# Autodesk Inventor assembly: robot_over_all5
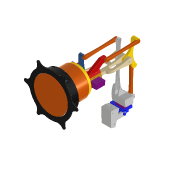
[picture p0: Inventor's stored thumbnail of the model, 180x180]
Saved by Autodesk Inventor 2022.6 (Build 266554000, 554)
## iProperties
Created: 2025-03-10
Part Number: robot_over_all5
Document SubType Name: Assembly
Designer: rugby
Author: rugby
## Documents named in this file (21)
- C:\Users\rugby\Desktop\パンケーキFA工場\ロボットアーム_機械設計\垂直多関節リンクロボット\robot_over_all5.iam
- C:\Users\rugby\Desktop\パンケーキFA工場\ロボットアーム_機械設計\垂直多関節リンクロボット\base\base_02.ipt
- C:\Users\rugby\Desktop\パンケーキFA工場\ロボットアーム_機械設計\垂直多関節リンクロボット\base\base_holderTamTam_02.ipt
- C:\Users\rugby\Desktop\パンケーキFA工場\ロボットアーム_機械設計\ServoMotor(20kg・cm)\ServoMotor(20kg・cm).ipt
- C:\Users\rugby\Desktop\パンケーキFA工場\ロボットアーム_機械設計\垂直多関節リンクロボット\base\roofparts_support_upper2.ipt
- C:\Users\rugby\Desktop\パンケーキFA工場\ロボットアーム_機械設計\垂直多関節リンクロボット\base\joint1_roofparts.ipt
- C:\Users\rugby\Desktop\パンケーキFA工場\ロボットアーム_機械設計\ServoMotor(20kg・cm)\ServoMotor_Hone1.ipt
- C:\Users\rugby\Desktop\パンケーキFA工場\ロボットアーム_機械設計\垂直多関節リンクロボット\base\j2_j3_support3.ipt
- C:\Users\rugby\Desktop\パンケーキFA工場\平行リンクロボットCAD\servo_cover2.ipt
- C:\Users\rugby\Desktop\パンケーキFA工場\ロボットアーム_機械設計\垂直多関節リンクロボット\link\arm_42.ipt
- C:\Users\rugby\Desktop\パンケーキFA工場\ロボットアーム_機械設計\ServoMotor(20kg・cm)\ServoMotor_Hone2.ipt
- C:\Users\rugby\Desktop\パンケーキFA工場\ロボットアーム_機械設計\垂直多関節リンクロボット\link\arm_53.ipt
- C:\Users\rugby\Desktop\パンケーキFA工場\ロボットアーム_機械設計\垂直多関節リンクロボット\link\arm_51.ipt
- C:\Users\rugby\Desktop\パンケーキFA工場\ロボットアーム_機械設計\垂直多関節リンクロボット\link\arm_64.ipt
- C:\Users\rugby\Desktop\パンケーキFA工場\ロボットアーム_機械設計\垂直多関節リンクロボット\link\arm_55.ipt
- C:\Users\rugby\Desktop\パンケーキFA工場\ロボットアーム_機械設計\垂直多関節リンクロボット\link\arm_63.ipt
- C:\Users\rugby\Desktop\パンケーキFA工場\ロボットアーム_機械設計\垂直多関節リンクロボット\wrist1\j4_cover 2.ipt
- C:\Users\rugby\Desktop\パンケーキFA工場\ロボットアーム_機械設計\垂直多関節リンクロボット\wrist2\joint5_cover 2.ipt
- C:\Users\rugby\Desktop\パンケーキFA工場\ロボットアーム_機械設計\SG90_servoMotor\SG90_MainBody.ipt
- C:\Users\rugby\Desktop\パンケーキFA工場\ロボットアーム_機械設計\垂直多関節リンクロボット\endeffecta\fri_gripper_left2.ipt
- C:\Users\rugby\Desktop\パンケーキFA工場\ロボットアーム_機械設計\垂直多関節リンクロボット\endeffecta\fri_gripper_right2.ipt
## Components (27 placed, 20 different names)
1. base_02:1 — メイト:1, フラッシュ:1, メイト:2, メイト:3, メイト:4, メイト:5, メイト:6
2. base_holderTamTam_02:1 — メイト:1, フラッシュ:1
3. ServoMotor(20kg・cm):1 — メイト:2, メイト:3, メイト:4, メイト:12, メイト:13
4. roofparts_support_upper2:1 — メイト:5, メイト:6
5. ServoMotor_Hone1:1 — メイト:9, メイト:10, メイト:11, メイト:13
6. joint1_roofparts:1 — メイト:9, メイト:10, メイト:11, メイト:12, メイト:14, メイト:15, メイト:16
7. j2_j3_support3:1 — メイト:14, メイト:15, メイト:16, メイト:19, メイト:20, メイト:21, メイト:22, メイト:24, メイト:25, メイト:26, メイト:27, メイト:28, メイト:29, メイト:30, メイト:31, メイト:32, メイト:48, メイト:49
8. ServoMotor(20kg・cm):2 — メイト:19, メイト:20, メイト:21, メイト:22, メイト:34, メイト:40
9. ServoMotor(20kg・cm):3 — メイト:26, メイト:27, メイト:28, メイト:33, メイト:39
10. servo_cover2:1 — メイト:30, メイト:31, メイト:32
11. servo_cover2:2 — メイト:24, メイト:25, メイト:29
12. arm_42:1 — メイト:35, メイト:36, メイト:37, メイト:41, メイト:42
13. ServoMotor_Hone2:1 — メイト:33, メイト:39, メイト:43, メイト:44
14. ServoMotor_Hone2:2 — メイト:34, メイト:35, メイト:36, メイト:37, メイト:40
15. arm_53:1 — メイト:41, メイト:42, メイト:45, メイト:47
16. arm_51:1 — メイト:43, メイト:44, メイト:46, メイト:51, メイト:54
17. arm_64:1 — メイト:45, メイト:46, メイト:47, メイト:55
18. arm_53:2 — メイト:48, メイト:49, メイト:50
19. arm_55:1 — メイト:50, メイト:51, メイト:52, メイト:53, メイト:54
20. arm_63:1 — メイト:52, メイト:53, メイト:56, メイト:57
21. j4_cover 2:1 — メイト:55, メイト:56, メイト:57, メイト:65, メイト:66, メイト:67
22. joint5_cover 2:1 — メイト:70, メイト:71, メイト:73, メイト:75
23. SG90_MainBody:1 — メイト:72, メイト:74
24. fri_gripper_left2:1 — メイト:73, メイト:75
25. fri_gripper_right2:1 — メイト:72, メイト:74
26. ServoMotor(20kg・cm):4 — メイト:65, メイト:66, メイト:67, メイト:68, メイト:69, メイト:70
27. ServoMotor_Hone1:2 — メイト:68, メイト:69, メイト:71
## Relationships (66: Mate 65, Flush 1)
- メイト:1 [Mate]: base_02:1 ↔ base_holderTamTam_02:1
- フラッシュ:1 [Flush]: base_02:1 ↔ base_holderTamTam_02:1
- メイト:2 [Mate]: base_02:1 ↔ ServoMotor(20kg・cm):1
- メイト:3 [Mate] (0.5 mm): base_02:1 ↔ ServoMotor(20kg・cm):1
- メイト:4 [Mate]: base_02:1 ↔ ServoMotor(20kg・cm):1
- メイト:5 [Mate]: base_02:1 ↔ roofparts_support_upper2:1
- メイト:6 [Mate]: base_02:1 ↔ roofparts_support_upper2:1
- メイト:9 [Mate]: ServoMotor_Hone1:1 ↔ joint1_roofparts:1
- メイト:10 [Mate] (0.4 mm): ServoMotor_Hone1:1 ↔ joint1_roofparts:1
- メイト:11 [Mate]: ServoMotor_Hone1:1 ↔ joint1_roofparts:1
- メイト:12 [Mate]: ServoMotor(20kg・cm):1 ↔ joint1_roofparts:1
- メイト:13 [Mate]: ServoMotor(20kg・cm):1 ↔ ServoMotor_Hone1:1
- メイト:14 [Mate]: joint1_roofparts:1 ↔ j2_j3_support3:1
- メイト:15 [Mate]: joint1_roofparts:1 ↔ j2_j3_support3:1
- メイト:16 [Mate]: joint1_roofparts:1 ↔ j2_j3_support3:1
- メイト:19 [Mate]: j2_j3_support3:1 ↔ ServoMotor(20kg・cm):2
- メイト:20 [Mate]: j2_j3_support3:1 ↔ ServoMotor(20kg・cm):2
- メイト:21 [Mate]: j2_j3_support3:1 ↔ ServoMotor(20kg・cm):2
- メイト:22 [Mate]: j2_j3_support3:1 ↔ ServoMotor(20kg・cm):2
- メイト:24 [Mate]: j2_j3_support3:1 ↔ servo_cover2:2
- メイト:25 [Mate]: j2_j3_support3:1 ↔ servo_cover2:2
- メイト:26 [Mate]: j2_j3_support3:1 ↔ ServoMotor(20kg・cm):3
- メイト:27 [Mate]: j2_j3_support3:1 ↔ ServoMotor(20kg・cm):3
- メイト:28 [Mate]: j2_j3_support3:1 ↔ ServoMotor(20kg・cm):3
- メイト:29 [Mate]: j2_j3_support3:1 ↔ servo_cover2:2
- メイト:30 [Mate]: j2_j3_support3:1 ↔ servo_cover2:1
- メイト:31 [Mate]: j2_j3_support3:1 ↔ servo_cover2:1
- メイト:32 [Mate]: j2_j3_support3:1 ↔ servo_cover2:1
- メイト:33 [Mate]: ServoMotor(20kg・cm):3 ↔ ServoMotor_Hone2:1
- メイト:34 [Mate]: ServoMotor(20kg・cm):2 ↔ ServoMotor_Hone2:2
- メイト:35 [Mate]: arm_42:1 ↔ ServoMotor_Hone2:2
- メイト:36 [Mate] (0.5 mm): arm_42:1 ↔ ServoMotor_Hone2:2
- メイト:37 [Mate]: arm_42:1 ↔ ServoMotor_Hone2:2
- メイト:39 [Mate] (1 mm): ServoMotor(20kg・cm):3 ↔ ServoMotor_Hone2:1
- メイト:40 [Mate] (1 mm): ServoMotor(20kg・cm):2 ↔ ServoMotor_Hone2:2
- メイト:41 [Mate]: arm_42:1 ↔ arm_53:1
- メイト:42 [Mate]: arm_42:1 ↔ arm_53:1
- メイト:43 [Mate]: ServoMotor_Hone2:1 ↔ arm_51:1
- メイト:44 [Mate]: ServoMotor_Hone2:1 ↔ arm_51:1
- メイト:45 [Mate]: arm_53:1 ↔ arm_64:1
- メイト:46 [Mate]: arm_51:1 ↔ arm_64:1
- メイト:47 [Mate]: arm_53:1 ↔ arm_64:1
- メイト:48 [Mate]: j2_j3_support3:1 ↔ arm_53:2
- メイト:49 [Mate]: j2_j3_support3:1 ↔ arm_53:2
- メイト:50 [Mate]: arm_53:2 ↔ arm_55:1
- メイト:51 [Mate]: arm_51:1 ↔ arm_55:1
- メイト:52 [Mate]: arm_55:1 ↔ arm_63:1
- メイト:53 [Mate]: arm_55:1 ↔ arm_63:1
- メイト:54 [Mate]: arm_51:1 ↔ arm_55:1
- メイト:55 [Mate]: arm_64:1 ↔ j4_cover 2:1
- メイト:56 [Mate]: arm_63:1 ↔ j4_cover 2:1
- メイト:57 [Mate]: arm_63:1 ↔ j4_cover 2:1
- [Mate]: joint5_cover 2:1 ↔ SG90_MainBody:1
- [Mate]: joint5_cover 2:1 ↔ SG90_MainBody:1
- [Mate]: joint5_cover 2:1 ↔ SG90_MainBody:1
- メイト:65 [Mate]: j4_cover 2:1 ↔ ServoMotor(20kg・cm):4
- メイト:66 [Mate]: j4_cover 2:1 ↔ ServoMotor(20kg・cm):4
- メイト:67 [Mate]: j4_cover 2:1 ↔ ServoMotor(20kg・cm):4
- メイト:68 [Mate]: ServoMotor(20kg・cm):4 ↔ ServoMotor_Hone1:2
- メイト:69 [Mate]: ServoMotor(20kg・cm):4 ↔ ServoMotor_Hone1:2
- メイト:70 [Mate]: joint5_cover 2:1 ↔ ServoMotor(20kg・cm):4
- メイト:71 [Mate]: joint5_cover 2:1 ↔ ServoMotor_Hone1:2
- メイト:72 [Mate]: SG90_MainBody:1 ↔ fri_gripper_right2:1
- メイト:73 [Mate]: joint5_cover 2:1 ↔ fri_gripper_left2:1
- メイト:74 [Mate]: SG90_MainBody:1 ↔ fri_gripper_right2:1
- メイト:75 [Mate]: joint5_cover 2:1 ↔ fri_gripper_left2:1
